# Autodesk Inventor assembly: CoreXY Idler 4040 Assembly Right V2
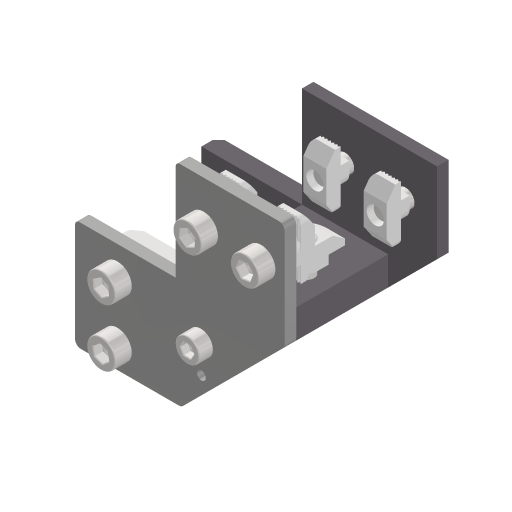
[picture p0: Inventor's stored thumbnail of the model, 512x512]
Saved by Autodesk Inventor 2023.2 (Build 272271000, 271)
## iProperties
Created: 2023-11-27
Part Number: CoreXY Idler 4040 Assembly Right V2
Document SubType Name: Assembly
Designer: Nils Bade
Author: Nils Bade
## Documents named in this file (13)
- C:\Users\nilsb\Documents\Inventor\Projektarbeit-Bade\RatRig_Bade\CoreXY Idler 4040 Assembly Right V2.iam
- C:\Users\nilsb\Documents\Inventor\Projektarbeit-Bade\RatRig_modified\Idler Plate for 4040.ipt
- C:\Users\nilsb\Documents\Inventor\Projektarbeit-Bade\RatRig_Standards\Hex Locking Nut - M5 v2.ipt
- C:\Users\nilsb\Documents\Inventor\Projektarbeit-Bade\RatRig_modified\T-NUT - DropIn 4040 SERIES - M6.ipt
- C:\Users\nilsb\Documents\Inventor\Projektarbeit-Bade\Schrauben\Cap Head Screw M6x16.ipt
- C:\Users\nilsb\Documents\Inventor\Projektarbeit-Bade\Schrauben\Cap Head Screw M6x12 v2.ipt
- C:\Users\nilsb\Documents\Inventor\Projektarbeit-Bade\Schrauben\Countersink Screw M6x14 v2.ipt
- C:\Users\nilsb\Documents\Inventor\Projektarbeit-Bade\RatRig_Standards\Mini Precision Shim - 8x5x1mm v2.ipt
- C:\Users\nilsb\Documents\Inventor\Projektarbeit-Bade\RatRig_Standards\Ball Bearing - F695ZZ v1.ipt
- C:\Users\nilsb\Documents\Inventor\Projektarbeit-Bade\RatRig_Standards\Ball Bearing - 695ZZ v1.ipt
- C:\Users\nilsb\Documents\Inventor\Projektarbeit-Bade\RatRig_Standards\Aluminium Spacer - 6mm v2.ipt
- C:\Users\nilsb\Documents\Inventor\Projektarbeit-Bade\RatRig_modified\xy Idler Right for 4040 V2.ipt
- C:\Users\nilsb\Documents\Inventor\Projektarbeit-Bade\Schrauben\Cap Head Screw M5x50.ipt
## Components (28 placed, 12 different names)
1. xy Idler Right for 4040 V2:1 — Passend:58, Passend:59
2. Idler Plate for 4040:1 — Passend:6, Passend:7, Passend:8, Passend:9, Winkel:4, Winkel:5, Winkel:6, Winkel:7, Passend:16, Passend:17, Passend:22, Passend:23, Passend:26, Passend:27, Passend:28, Passend:29, Passend:30, Passend:31, Passend:32, Passend:33, Passend:43
3. Cap Head Screw M5x50:1
4. Hex Locking Nut - M5 v2:1
5. T-NUT - DROP IN TYPE FOR 40 SERIES - M6:1
6. T-NUT - DROP IN TYPE FOR 40 SERIES - M6:2 — Passend:13
7. T-NUT - DROP IN TYPE FOR 40 SERIES - M6:3
8. T-NUT - DROP IN TYPE FOR 40 SERIES - M6:4
9. T-NUT - DROP IN TYPE FOR 40 SERIES - M6:6 — Passend:8, Winkel:5, Passend:17
10. T-NUT - DROP IN TYPE FOR 40 SERIES - M6:7 — Passend:9, Winkel:4, Passend:16
11. T-NUT - DROP IN TYPE FOR 40 SERIES - M6:8 — Passend:6, Winkel:7, Passend:22
12. T-NUT - DROP IN TYPE FOR 40 SERIES - M6:9 — Passend:7, Winkel:6, Passend:23
13. Cap Head Screw M6x16:1 — Passend:58, Passend:59
14. Cap Head Screw M6x12 v2:1 — Passend:29, Passend:33
15. Cap Head Screw M6x12 v2:2 — Passend:28, Passend:32
16. Cap Head Screw M6x12 v2:3 — Passend:26, Passend:30
17. Cap Head Screw M6x12 v2:4 — Passend:27, Passend:31
18. Countersink Screw M6x14 v2:1 — Passend:13
19. Countersink Screw M6x14 v2:2
20. Countersink Screw M6x14 v2:4
21. Mini Precision Shim - 8x5x1mm v2:1 — Passend:43, Passend:45
22. Mini Precision Shim - 8x5x1mm v2:2 — Passend:49, Passend:51
23. Mini Precision Shim - 8x5x1mm v2:3 — Passend:57
24. Ball Bearing - F695ZZ v1:1 — Passend:55, Passend:57
25. Ball Bearing - F695ZZ v1:2 — Passend:51, Passend:53
26. Ball Bearing - 695ZZ v1:1 — Passend:53, Passend:55
27. Aluminium Spacer - 6mm v2:1 — Passend:45, Passend:47
28. Aluminium Spacer - 6mm v2:2 — Passend:47, Passend:49
## Relationships (64: Mate 53, Angle 9, Flush 2)
- [Flush]: xy Idler Right for 4040 V2:1 ↔ Idler Plate for 4040:1
- [Flush]: xy Idler Right for 4040 V2:1 ↔ Idler Plate for 4040:1
- [Mate]: xy Idler Right for 4040 V2:1 ↔ Idler Plate for 4040:1
- [Mate]: Idler Plate for 4040:1 ↔ Cap Head Screw M5x50:1
- [Mate]: Idler Plate for 4040:1 ↔ Cap Head Screw M5x50:1
- [Mate]: Cap Head Screw M5x50:1 ↔ Hex Locking Nut - M5 v2:1
- [Mate]: xy Idler Right for 4040 V2:1 ↔ Hex Locking Nut - M5 v2:1
- [Angle] (0 deg): xy Idler Right for 4040 V2:1 ↔ Hex Locking Nut - M5 v2:1
- Passend:6 [Mate]: Idler Plate for 4040:1 ↔ T-NUT - DROP IN TYPE FOR 40 SERIES - M6:8
- Passend:7 [Mate]: Idler Plate for 4040:1 ↔ T-NUT - DROP IN TYPE FOR 40 SERIES - M6:9
- Passend:8 [Mate]: Idler Plate for 4040:1 ↔ T-NUT - DROP IN TYPE FOR 40 SERIES - M6:6
- Passend:9 [Mate]: Idler Plate for 4040:1 ↔ T-NUT - DROP IN TYPE FOR 40 SERIES - M6:7
- [Mate]: xy Idler Right for 4040 V2:1 ↔ T-NUT - DROP IN TYPE FOR 40 SERIES - M6:4
- [Mate]: xy Idler Right for 4040 V2:1 ↔ T-NUT - DROP IN TYPE FOR 40 SERIES - M6:3
- Passend:13 [Mate]: T-NUT - DROP IN TYPE FOR 40 SERIES - M6:2 ↔ Countersink Screw M6x14 v2:1
- [Angle] (0 deg): xy Idler Right for 4040 V2:1 ↔ T-NUT - DROP IN TYPE FOR 40 SERIES - M6:4
- Winkel:4 [Angle] (0 deg): Idler Plate for 4040:1 ↔ T-NUT - DROP IN TYPE FOR 40 SERIES - M6:7
- Winkel:5 [Angle] (0 deg): Idler Plate for 4040:1 ↔ T-NUT - DROP IN TYPE FOR 40 SERIES - M6:6
- Winkel:6 [Angle] (0 deg): Idler Plate for 4040:1 ↔ T-NUT - DROP IN TYPE FOR 40 SERIES - M6:9
- Winkel:7 [Angle] (0 deg): Idler Plate for 4040:1 ↔ T-NUT - DROP IN TYPE FOR 40 SERIES - M6:8
- [Angle] (0 deg): xy Idler Right for 4040 V2:1 ↔ T-NUT - DROP IN TYPE FOR 40 SERIES - M6:1
- [Mate] (5.5 mm): xy Idler Right for 4040 V2:1 ↔ T-NUT - DROP IN TYPE FOR 40 SERIES - M6:4
- Passend:16 [Mate] (5.5 mm): Idler Plate for 4040:1 ↔ T-NUT - DROP IN TYPE FOR 40 SERIES - M6:7
- Passend:17 [Mate] (5.5 mm): Idler Plate for 4040:1 ↔ T-NUT - DROP IN TYPE FOR 40 SERIES - M6:6
- [Mate] (5.5 mm): xy Idler Right for 4040 V2:1 ↔ T-NUT - DROP IN TYPE FOR 40 SERIES - M6:1
- [Mate]: xy Idler Right for 4040 V2:1 ↔ T-NUT - DROP IN TYPE FOR 40 SERIES - M6:1
- [Angle] (0 deg): xy Idler Right for 4040 V2:1 ↔ T-NUT - DROP IN TYPE FOR 40 SERIES - M6:3
- [Angle] (0 deg): xy Idler Right for 4040 V2:1 ↔ T-NUT - DROP IN TYPE FOR 40 SERIES - M6:2
- [Mate] (5.5 mm): xy Idler Right for 4040 V2:1 ↔ T-NUT - DROP IN TYPE FOR 40 SERIES - M6:3
- [Mate] (5.5 mm): xy Idler Right for 4040 V2:1 ↔ T-NUT - DROP IN TYPE FOR 40 SERIES - M6:2
- Passend:22 [Mate] (5.5 mm): Idler Plate for 4040:1 ↔ T-NUT - DROP IN TYPE FOR 40 SERIES - M6:8
- Passend:23 [Mate] (5.5 mm): Idler Plate for 4040:1 ↔ T-NUT - DROP IN TYPE FOR 40 SERIES - M6:9
- Passend:26 [Mate]: Idler Plate for 4040:1 ↔ Cap Head Screw M6x12 v2:3
- Passend:27 [Mate]: Idler Plate for 4040:1 ↔ Cap Head Screw M6x12 v2:4
- Passend:28 [Mate]: Idler Plate for 4040:1 ↔ Cap Head Screw M6x12 v2:2
- Passend:29 [Mate]: Idler Plate for 4040:1 ↔ Cap Head Screw M6x12 v2:1
- Passend:30 [Mate]: Idler Plate for 4040:1 ↔ Cap Head Screw M6x12 v2:3
- Passend:31 [Mate]: Idler Plate for 4040:1 ↔ Cap Head Screw M6x12 v2:4
- Passend:32 [Mate]: Idler Plate for 4040:1 ↔ Cap Head Screw M6x12 v2:2
- Passend:33 [Mate]: Idler Plate for 4040:1 ↔ Cap Head Screw M6x12 v2:1
- [Mate]: xy Idler Right for 4040 V2:1 ↔ Countersink Screw M6x14 v2:1
- [Mate]: xy Idler Right for 4040 V2:1 ↔ Countersink Screw M6x14 v2:2
- [Mate]: xy Idler Right for 4040 V2:1 ↔ Countersink Screw M6x14 v2:4
- [Mate]: xy Idler Right for 4040 V2:1 ↔ Countersink Screw M6x14 v2:1
- [Mate]: xy Idler Right for 4040 V2:1 ↔ Countersink Screw M6x14 v2:2
- [Mate]: xy Idler Right for 4040 V2:1 ↔ Countersink Screw M6x14 v2:4
- [Mate]: Cap Head Screw M5x50:1 ↔ Mini Precision Shim - 8x5x1mm v2:1
- Passend:43 [Mate]: Idler Plate for 4040:1 ↔ Mini Precision Shim - 8x5x1mm v2:1
- [Mate]: Cap Head Screw M5x50:1 ↔ Aluminium Spacer - 6mm v2:1
- Passend:45 [Mate]: Mini Precision Shim - 8x5x1mm v2:1 ↔ Aluminium Spacer - 6mm v2:1
- [Mate]: Cap Head Screw M5x50:1 ↔ Aluminium Spacer - 6mm v2:2
- Passend:47 [Mate]: Aluminium Spacer - 6mm v2:1 ↔ Aluminium Spacer - 6mm v2:2
- [Mate]: Cap Head Screw M5x50:1 ↔ Mini Precision Shim - 8x5x1mm v2:2
- Passend:49 [Mate]: Mini Precision Shim - 8x5x1mm v2:2 ↔ Aluminium Spacer - 6mm v2:2
- [Mate]: Cap Head Screw M5x50:1 ↔ Ball Bearing - F695ZZ v1:2
- Passend:51 [Mate]: Mini Precision Shim - 8x5x1mm v2:2 ↔ Ball Bearing - F695ZZ v1:2
- [Mate]: Cap Head Screw M5x50:1 ↔ Ball Bearing - 695ZZ v1:1
- Passend:53 [Mate]: Ball Bearing - F695ZZ v1:2 ↔ Ball Bearing - 695ZZ v1:1
- [Mate]: Cap Head Screw M5x50:1 ↔ Ball Bearing - F695ZZ v1:1
- Passend:55 [Mate]: Ball Bearing - F695ZZ v1:1 ↔ Ball Bearing - 695ZZ v1:1
- [Mate]: Cap Head Screw M5x50:1 ↔ Mini Precision Shim - 8x5x1mm v2:3
- Passend:57 [Mate]: Mini Precision Shim - 8x5x1mm v2:3 ↔ Ball Bearing - F695ZZ v1:1
- Passend:58 [Mate]: xy Idler Right for 4040 V2:1 ↔ Cap Head Screw M6x16:1
- Passend:59 [Mate]: xy Idler Right for 4040 V2:1 ↔ Cap Head Screw M6x16:1
